# Autodesk Inventor assembly: ASY MSC 203 RIGHT BOARD
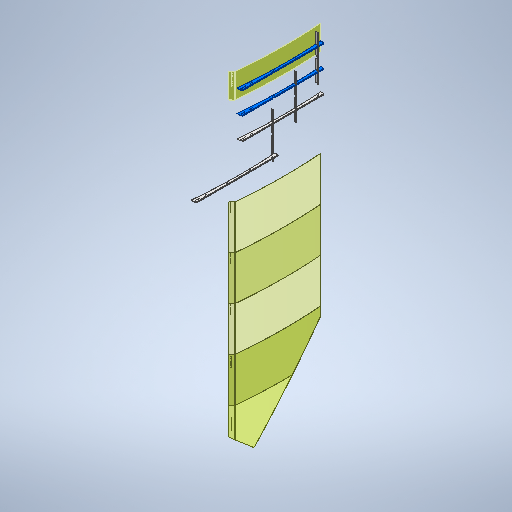
[picture p0: Inventor's stored thumbnail of the model, 512x512]
Saved by Autodesk Inventor 2025 (Build 290162010, 162A)
## iProperties
Created: 2024-07-22
Part Number: ASY MSC 203 RIGHT BOARD
Document SubType Name: Assembly
Designer: pokla
Author: pokla
## Documents named in this file (9)
- C:\Users\admin\YandexDisk-badmisterfox\домашниий пк\Inventor\Manturovo\Manturovo_Se-clar\ASY MSC 203 RIGHT BOARD.iam
- C:\Users\admin\YandexDisk-badmisterfox\домашниий пк\Inventor\Manturovo\Manturovo_Se-clar\MSC 052 rib board.ipt
- C:\Users\admin\YandexDisk-badmisterfox\домашниий пк\Inventor\Manturovo\Manturovo_Se-clar\MSC 024 sheet board main.ipt
- C:\Users\admin\YandexDisk-badmisterfox\домашниий пк\Inventor\Manturovo\Manturovo_Se-clar\MSC 023 sheet board.ipt
- C:\Users\admin\YandexDisk-badmisterfox\домашниий пк\Inventor\Manturovo\Manturovo_Se-clar\MSC 025.2 sheet board withers.ipt
- C:\Users\admin\YandexDisk-badmisterfox\домашниий пк\Inventor\Manturovo\Manturovo_Se-clar\MSC 063 stringer BOARD  #.ipt
- C:\Users\admin\YandexDisk-badmisterfox\домашниий пк\Inventor\Manturovo\Manturovo_Se-clar\MSC 064 stringer BOARD  ##.ipt
- C:\Users\admin\YandexDisk-badmisterfox\домашниий пк\Inventor\Manturovo\Manturovo_Se-clar\MSC 027.2 sheet board withers 4.ipt
- C:\Users\admin\YandexDisk-badmisterfox\домашниий пк\Inventor\Manturovo\Manturovo_Se-clar\MSC 065 stringer BOARD  ###.ipt
## Components (15 placed, 9 different names)
1. MSC 052 rib board.ipt:1 — Rigid:43
2. MSC 024 sheet board main.ipt:6 — Rigid:42
3. MSC 024 sheet board main.ipt:7
4. MSC 024 sheet board main.ipt:8
5. MSC 024 sheet board main.ipt:9
6. MSC 024 sheet board main.ipt:10
7. MSC 023 sheet board.ipt:2
8. MSC 052 rib board.ipt:4 — Rigid:44, Rigid:45
9. MSC 025.2 sheet board withers:1 — Rigid:42, Rigid:46
10. MSC 063 stringer BOARD  #:1 — Rigid:43, Rigid:44
11. MSC 064 stringer BOARD  ##:1 — Rigid:45, Rigid:47
12. MSC 027.2 sheet board withers 4:1 — Rigid:46
13. MSC 052 rib board:3 — Rigid:47, Rigid:48
14. MSC 065 stringer BOARD  ###:1 — Rigid:48
15. MSC 052 rib board:5
## Relationships (12: WeldJoint 12)
- [WeldJoint]: MSC 024 sheet board main.ipt:6 ↔ MSC 024 sheet board main.ipt:7
- [WeldJoint]: MSC 024 sheet board main.ipt:7 ↔ MSC 024 sheet board main.ipt:8
- [WeldJoint]: MSC 024 sheet board main.ipt:8 ↔ MSC 024 sheet board main.ipt:9
- [WeldJoint]: MSC 024 sheet board main.ipt:9 ↔ MSC 024 sheet board main.ipt:10
- [WeldJoint]: MSC 024 sheet board main.ipt:10 ↔ MSC 023 sheet board.ipt:2
- Rigid:42 [WeldJoint]: MSC 024 sheet board main.ipt:6 ↔ MSC 025.2 sheet board withers:1
- Rigid:43 [WeldJoint] (2 mm): MSC 052 rib board.ipt:1 ↔ MSC 063 stringer BOARD  #:1
- Rigid:44 [WeldJoint] (2 mm): MSC 052 rib board.ipt:4 ↔ MSC 063 stringer BOARD  #:1
- Rigid:45 [WeldJoint] (2 mm): MSC 052 rib board.ipt:4 ↔ MSC 064 stringer BOARD  ##:1
- Rigid:46 [WeldJoint]: MSC 025.2 sheet board withers:1 ↔ MSC 027.2 sheet board withers 4:1
- Rigid:47 [WeldJoint] (2 mm): MSC 064 stringer BOARD  ##:1 ↔ MSC 052 rib board:3
- Rigid:48 [WeldJoint]: MSC 052 rib board:3 ↔ MSC 065 stringer BOARD  ###:1
## Named parameters: d230_d194 = 0 mm, d231_d195 = 0 mm, d232_d160 = 0 mm, d233_d161 = 0 mm
